# Autodesk Inventor assembly: Arduino_Oktagon
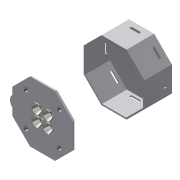
[picture p0: Inventor's stored thumbnail of the model, 180x180]
Saved by Autodesk Inventor 2018.2 (Build 222227000, 227)
## iProperties
Company: Fraunhofer ILT
Created: 2018-10-01
Part Number: Arduino_Oktagon
Material: geeigneten Werkstoff auswählen !
Document SubType Name: Assembly
Designer: N.Grubert
Title: =Description
Author: N.Grubert
## Documents named in this file (3)
- C:\Users\GRUBERT\Documents\COSIMA-Laserstar\CAD\Arduino_Oktagon.iam
- C:\Users\GRUBERT\Documents\COSIMA-Laserstar\CAD\Oktagon.ipt
- C:\Users\GRUBERT\Documents\COSIMA-Laserstar\CAD\DeckelParabol.iam
## Components (2 placed, 2 different names)
1. Oktagon:1 — Passend:1, Passend:2, Passend:3, Passend:4, Fluchtend:1, Fluchtend:2, Passend:5
2. DeckelParabol:1 [sub-assembly] — Fluchtend:1, Fluchtend:2, Passend:5
## Relationships (7: Mate 5, Flush 2)
- Passend:1 [Mate]: Oktagon:1
- Passend:2 [Mate]: Oktagon:1
- Passend:3 [Mate]: Oktagon:1
- Passend:4 [Mate]: Oktagon:1
- Fluchtend:1 [Flush]: Oktagon:1 ↔ DeckelParabol:1
- Fluchtend:2 [Flush]: Oktagon:1 ↔ DeckelParabol:1
- Passend:5 [Mate]: Oktagon:1 ↔ DeckelParabol:1
